# Autodesk Inventor assembly: full
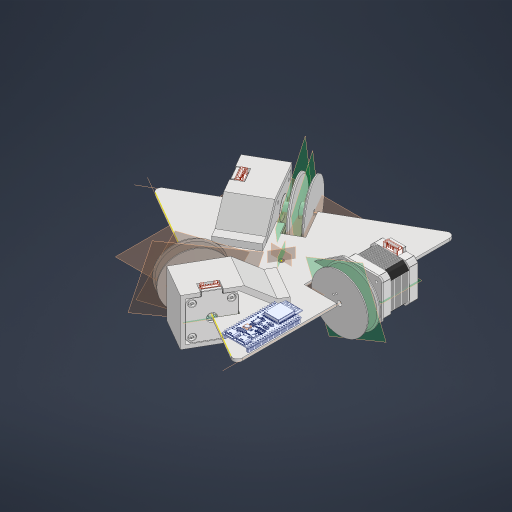
[picture p0: Inventor's stored thumbnail of the model, 512x512]
Saved by Autodesk Inventor 2024 (Build 280153000, 153)
## iProperties
Created: 2026-03-23
Part Number: full
Document SubType Name: Assembly
Designer: schar
Author: schar
## Documents named in this file (6)
- C:\Users\schar\Desktop\FloatingFace\models\full.iam
- C:\Users\schar\Desktop\FloatingFace\models\baseplate.ipt
- C:\Users\schar\Desktop\FloatingFace\models\spool.ipt
- C:\Users\schar\Desktop\FloatingFace\models\17HS4401S_Stepper_Motor\17HS4401S_Stepper_Motor.iam
- C:\Users\schar\Desktop\FloatingFace\models\esp32-s3-wroom-1-1.snapshot.2\ESP32-S3-WROOM-1\ESP32-S3-WROOM-1.iam
- C:\Users\schar\Desktop\FloatingFace\models\nema_brackets_and_lineguides.ipt
## Components (10 placed, 5 different names)
1. baseplate:1 — Mate:1, Mate:2, Mate:3, Mate:6, Mate:11, Mate:12, Flush:1, Mate:13, Mate:14, Mate:15, Flush:2, Flush:3, Flush:11
2. spool:1 — Mate:1, Mate:2, Mate:4, Mate:5
3. 17HS4401S_Stepper_Motor:1 [sub-assembly] — Mate:3, Mate:4, Mate:5
4. ESP32-S3-WROOM-1:1 [sub-assembly] — Mate:6
5. spool:2
6. 17HS4401S_Stepper_Motor:4 [sub-assembly] — Mate:14, Mate:15, Flush:2, Mate:16, Mate:17
7. spool:3 — Mate:11, Flush:4
8. 17HS4401S_Stepper_Motor:5 [sub-assembly] — Mate:12, Flush:1, Mate:13
9. nema_brackets_and_lineguides:1 — Flush:3, Flush:4, Flush:10
10. nema_brackets_and_lineguides:2 — Mate:16, Flush:11, Mate:17, Flush:12
## Relationships (24: Mate 17, Flush 7)
- Mate:1: baseplate:1 ↔ spool:1
- Mate:2: baseplate:1 ↔ spool:1
- Mate:3: baseplate:1 ↔ 17HS4401S_Stepper_Motor:1
- Mate:4: spool:1 ↔ 17HS4401S_Stepper_Motor:1
- Mate:5: spool:1 ↔ 17HS4401S_Stepper_Motor:1
- Mate:6: baseplate:1 ↔ ESP32-S3-WROOM-1:1
- [Mate]: spool:2 ↔ 17HS4401S_Stepper_Motor:4
- [Mate]: spool:2 ↔ 17HS4401S_Stepper_Motor:4
- [Mate]: spool:3 ↔ 17HS4401S_Stepper_Motor:5
- [Mate]: spool:3 ↔ 17HS4401S_Stepper_Motor:5
- Mate:11: baseplate:1 ↔ spool:3
- Mate:12: baseplate:1 ↔ 17HS4401S_Stepper_Motor:5
- Flush:1: baseplate:1 ↔ 17HS4401S_Stepper_Motor:5
- Mate:13: baseplate:1 ↔ 17HS4401S_Stepper_Motor:5
- Mate:14: baseplate:1 ↔ 17HS4401S_Stepper_Motor:4
- Mate:15: baseplate:1 ↔ 17HS4401S_Stepper_Motor:4
- Flush:2: baseplate:1 ↔ 17HS4401S_Stepper_Motor:4
- Flush:3: baseplate:1 ↔ nema_brackets_and_lineguides:1
- Flush:4 (2 mm): spool:3 ↔ nema_brackets_and_lineguides:1
- Flush:10: nema_brackets_and_lineguides:1
- Mate:16: 17HS4401S_Stepper_Motor:4 ↔ nema_brackets_and_lineguides:2
- Flush:11: baseplate:1 ↔ nema_brackets_and_lineguides:2
- Mate:17: 17HS4401S_Stepper_Motor:4 ↔ nema_brackets_and_lineguides:2
- Flush:12: nema_brackets_and_lineguides:2
## Named parameters: d8_d5 = 0 mm, d9_d6 = 0 mm, d10_d5 = 0 mm, d11_d6 = 0 mm
